# Autodesk Inventor assembly: LeadScrewNutClamp
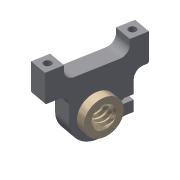
[picture p0: Inventor's stored thumbnail of the model, 180x180]
Saved by Autodesk Inventor 2018 (Build 220112000, 112)
## iProperties
Created: 2017-12-09
Part Number: LeadScrewNutClamp
Document SubType Name: Assembly
Designer: ball
Author: ball
## Documents named in this file (3)
- C:\FTC\FTC8863CAD\2017Robot\LeadScrewNutClamp.iam
- C:\FTC\FTC8863CAD\Actobotics\545 parts\545314.ipt
- C:\FTC\FTC8863CAD\Actobotics\585 parts\585546.ipt
## Components (2 placed, 2 different names)
1. 545314:1
2. 585546:1
## Relationships (2: Mate 1, Flush 1)
- [Mate]: 545314:1 ↔ 585546:1
- [Flush] (-3.175 mm): 545314:1 ↔ 585546:1
